# Autodesk Inventor assembly: prostkatna waska niska kwadraty v2
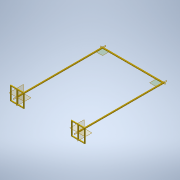
[picture p0: Inventor's stored thumbnail of the model, 180x180]
Saved by Autodesk Inventor 2021 (Build 250183000, 183)
## iProperties
Created: 2024-04-18
Part Number: prostkatna waska niska kwadraty v2
Document SubType Name: Assembly
Designer: Michal
Author: Michal
## Documents named in this file (5)
- C:\Users\Michal\Documents\GitHub\PNW_PhotoBoothFrame_3D\prostkatna waska niska kwadraty v2.iam
- C:\Users\Michal\Documents\GitHub\PNW_PhotoBoothFrame_3D\Stopa v1.iam
- C:\Users\Michal\Documents\GitHub\PNW_PhotoBoothFrame_3D\Naroznik v2.iam
- C:\Users\Michal\Documents\GitHub\PNW_PhotoBoothFrame_3D\Przedluzka L2400.ipt
- C:\Users\Michal\Documents\GitHub\PNW_PhotoBoothFrame_3D\Przedluzka L1680.ipt
## Components (7 placed, 4 different names)
1. Stopa v1:1 [sub-assembly] — Flush:1, Flush:2, Flush:5, Flush:6, Mate:14
2. Stopa v1:2 [sub-assembly] — Flush:1, Flush:2, Flush:7
3. Naroznik v2:1 [sub-assembly] — Mate:11
4. Przedluzka L2400:1 — Mate:11, Flush:5, Flush:6, Mate:14
5. Przedluzka L1680:1 — Mate:13
6. Naroznik v2:2 [sub-assembly] — Mate:12, Mate:13
7. Przedluzka L2400:2 — Mate:12, Flush:7
## Relationships (21: Mate 14, Flush 7)
- Flush:1: Stopa v1:1 ↔ Stopa v1:2
- Flush:2: Stopa v1:1 ↔ Stopa v1:2
- [Mate]: Naroznik v2:1 ↔ Przedluzka L2400:1
- [Mate]: Naroznik v2:1 ↔ Przedluzka L2400:1
- [Flush]: Naroznik v2:1 ↔ Przedluzka L1680:1
- [Mate]: Naroznik v2:1 ↔ Przedluzka L1680:1
- [Mate]: Naroznik v2:1 ↔ Przedluzka L1680:1
- [Mate]: Naroznik v2:2 ↔ Przedluzka L2400:2
- [Mate]: Naroznik v2:2 ↔ Przedluzka L2400:2
- [Mate]: Naroznik v2:2 ↔ Przedluzka L2400:2
- [Flush]: Przedluzka L1680:1 ↔ Przedluzka L2400:2
- [Mate]: Przedluzka L1680:1 ↔ Naroznik v2:2
- [Mate]: Przedluzka L1680:1 ↔ Naroznik v2:2
- [Mate]: Naroznik v2:1 ↔ Przedluzka L2400:1
- Mate:11: Naroznik v2:1 ↔ Przedluzka L2400:1
- Mate:12: Naroznik v2:2 ↔ Przedluzka L2400:2
- Mate:13: Przedluzka L1680:1 ↔ Naroznik v2:2
- Flush:5: Stopa v1:1 ↔ Przedluzka L2400:1
- Flush:6: Stopa v1:1 ↔ Przedluzka L2400:1
- Flush:7: Stopa v1:2 ↔ Przedluzka L2400:2
- Mate:14: Stopa v1:1 ↔ Przedluzka L2400:1
